# Autodesk Inventor assembly: carkifelek
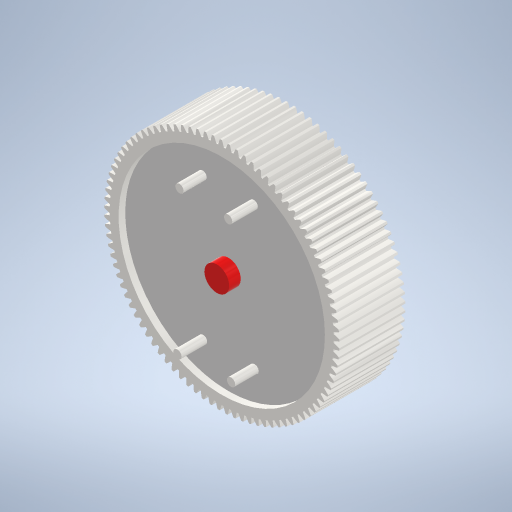
[picture p0: Inventor's stored thumbnail of the model, 512x512]
Saved by Autodesk Inventor 2023.2 (Build 272271000, 271)
## iProperties
Created: 2023-01-30
Part Number: carkifelek
Document SubType Name: Assembly
Designer: sarp1
Author: sarp1
## Documents named in this file (5)
- C:\Users\sarp1\Documents\hudson2022\otuzbir\YENI\carkifelek.iam
- C:\Users\sarp1\Documents\hudson2022\otuzbir\YENI\carkifelek\boyuk.ipt
- C:\Users\sarp1\Documents\hudson2022\otuzbir\YENI\carkifelek\kocuk.ipt
- C:\Users\sarp1\Documents\hudson2022\otuzbir\YENI\carkifelek\tutturgac.ipt
- C:\Users\sarp1\Documents\hudson2022\otuzbir\YENI\carkifelek\Design Accelerator\Spur Gears4.iam
## Components (9 placed, 4 different names)
1. Spur Gear2:1 — Mate:1, Mate:2, Mate:10, Mate:14, Mate:15, Rotation:2, Rotation:6, Rotation:8
2. Spur Gear1:1 — Mate:3, Mate:5, Rotation:1, Rotation:2
3. tutturgac:1 — Mate:1, Mate:2, Mate:3, Mate:4, Mate:5, Mate:6, Angle:1, Rotation:7, Rotation:8
4. Spur Gear1:2 — Mate:4, Mate:6, Rotation:4, Rotation:6
5. Spur Gear1:3 — Mate:9, Mate:12, Rotation:4, Rotation:5, Rotation:7
6. Spur Gear1:4 — Mate:8, Mate:13, Rotation:1, Rotation:3
7. tutturgac:2 — Mate:7, Mate:8, Mate:9, Mate:11, Mate:12, Mate:13
8. Spur Gear2:2 — Mate:7, Mate:10, Mate:11, Mate:14, Rotation:3, Rotation:5
9. dıs [sub-assembly] — Mate:15, Angle:1
## Relationships (24: Mate 15, RelateRotation 8, Angle 1)
- Mate:1: Spur Gear2:1 ↔ tutturgac:1
- Mate:2 (2 mm): Spur Gear2:1 ↔ tutturgac:1
- Mate:3: Spur Gear1:1 ↔ tutturgac:1
- Mate:4: tutturgac:1 ↔ Spur Gear1:2
- Mate:5 (15 mm): Spur Gear1:1 ↔ tutturgac:1
- Mate:6 (15 mm): tutturgac:1 ↔ Spur Gear1:2
- Mate:7: tutturgac:2 ↔ Spur Gear2:2
- Mate:8: Spur Gear1:4 ↔ tutturgac:2
- Mate:9: Spur Gear1:3 ↔ tutturgac:2
- Mate:10 (15 mm): Spur Gear2:1 ↔ Spur Gear2:2
- Mate:11 (2 mm): tutturgac:2 ↔ Spur Gear2:2
- Mate:12 (15 mm): Spur Gear1:3 ↔ tutturgac:2
- Mate:13 (15 mm): Spur Gear1:4 ↔ tutturgac:2
- Mate:14: Spur Gear2:1 ↔ Spur Gear2:2
- Mate:15: Spur Gear2:1 ↔ dıs
- Rotation:1 [RelateRotation] (1 ul): Spur Gear1:1 ↔ Spur Gear1:4
- Rotation:2 [RelateRotation] (0.333 ul): Spur Gear2:1 ↔ Spur Gear1:1
- Rotation:3 [RelateRotation] (3 ul): Spur Gear1:4 ↔ Spur Gear2:2
- Rotation:4 [RelateRotation] (1 ul): Spur Gear1:2 ↔ Spur Gear1:3
- Rotation:5 [RelateRotation] (3 ul): Spur Gear1:3 ↔ Spur Gear2:2
- Rotation:6 [RelateRotation] (3 ul): Spur Gear2:1 ↔ Spur Gear1:2
- Angle:1 (0 deg): tutturgac:1 ↔ dıs
- Rotation:7 [RelateRotation] (1 ul): tutturgac:1 ↔ Spur Gear1:3
- Rotation:8 [RelateRotation] (1 ul): Spur Gear2:1 ↔ tutturgac:1
